# Autodesk Inventor assembly: Base_test
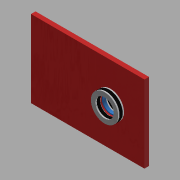
[picture p0: Inventor's stored thumbnail of the model, 180x180]
Saved by Autodesk Inventor 2019 (Build 230136000, 136)
## iProperties
Created: 2021-11-06
Part Number: Base_test
Document SubType Name: Assembly
Designer: Mohamed
Author: Mohamed
## Documents named in this file (4)
- F:\Semester 7\Design of mechatronics 1\SSCARA Robot\Base_test.iam
- F:\Semester 7\Design of mechatronics 1\SSCARA Robot\thrust bearing_40mm.iam
- F:\Semester 7\Design of mechatronics 1\SSCARA Robot\b_base cover_test 1.ipt
- F:\Semester 7\Design of mechatronics 1\SSCARA Robot\ball bearing 35mm.ipt
## Components (4 placed, 3 different names)
1. thrust bearing_40mm:1 [sub-assembly] — Mate:6, Mate:7
2. thrust bearing_40mm:2 [sub-assembly] — Mate:8, Mate:9
3. b_base cover_test 1:1 — Mate:1, Mate:5, Mate:6, Mate:7, Mate:8, Mate:9
4. ball bearing 35mm:1 — Mate:1, Mate:5
## Relationships (6: Mate 6)
- Mate:1: b_base cover_test 1:1 ↔ ball bearing 35mm:1
- Mate:5: b_base cover_test 1:1 ↔ ball bearing 35mm:1
- Mate:6: thrust bearing_40mm:1 ↔ b_base cover_test 1:1
- Mate:7: thrust bearing_40mm:1 ↔ b_base cover_test 1:1
- Mate:8: thrust bearing_40mm:2 ↔ b_base cover_test 1:1
- Mate:9: thrust bearing_40mm:2 ↔ b_base cover_test 1:1
